# Autodesk Inventor assembly: OGRobotAssembly
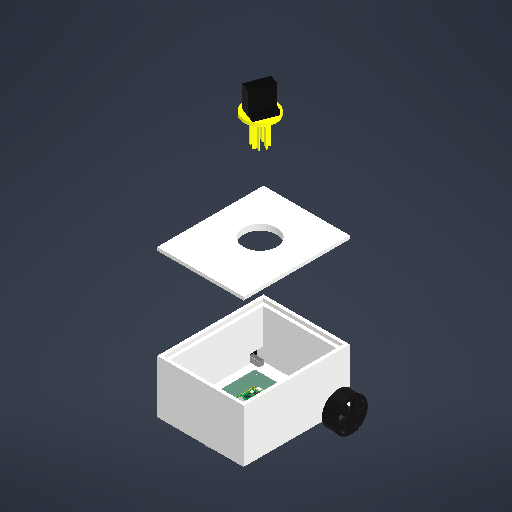
[picture p0: Inventor's stored thumbnail of the model, 512x512]
Saved by Autodesk Inventor 2027 (Build 310192060, 192F)
## iProperties
Created: 2026-07-04
Part Number: OGRobotAssembly
Document SubType Name: Assembly
Designer: machnach0
Author: machnach0
## Documents named in this file (9)
- C:\Users\machnach0\Documents\Inventor\Stardance Design Challenge\OGRobotAssembly.iam
- C:\Users\machnach0\Documents\Inventor\Stardance Design Challenge\OGRobotBase.ipt
- C:\Users\machnach0\Documents\Inventor\Stardance Design Challenge\OGRobotRoof.ipt
- C:\Users\machnach0\Documents\Inventor\Stardance Design Challenge\OGPlatform.ipt
- C:\Users\machnach0\Documents\Inventor\Stardance Design Challenge\OGWheel.ipt
- C:\Users\machnach0\Documents\Inventor\Stardance Design Challenge\OGGearMotor.ipt
- C:\Users\machnach0\Documents\Inventor\Stardance Design Challenge\OGCasterWheel.ipt
- C:\Users\machnach0\Documents\Inventor\Stardance Design Challenge\OGPCB.ipt
- C:\Users\machnach0\Documents\Inventor\Stardance Design Challenge\OGLiDAR.ipt
## Components (10 placed, 8 different names)
1. OGRobotBase:1 — Mate:1, Mate:2, Mate:9, Mate:10, Mate:11, Mate:12, Mate:13, Mate:14, Mate:15, Mate:16, Mate:17, Mate:18
2. OGRobotRoof:1 — Mate:1, Mate:2, Mate:4
3. OGPlatform:1 — Mate:4, Mate:19, Mate:20, Mate:21
4. OGWheel:1 — Mate:5, Mate:6, Mate:10
5. OGGearMotor:1 — Mate:5, Mate:6, Mate:9, Mate:11
6. OGWheel:2 — Mate:14
7. OGGearMotor:2 — Mate:12, Mate:13
8. OGCasterWheel:1 — Mate:15, Mate:16, Mate:17
9. OGPCB:1 — Mate:18
10. OGLiDAR:1 — Mate:19, Mate:20, Mate:21
## Relationships (20: Mate 20)
- Mate:1 (1.27 mm): OGRobotBase:1 ↔ OGRobotRoof:1
- Mate:2 (1.27 mm): OGRobotBase:1 ↔ OGRobotRoof:1
- Mate:4: OGRobotRoof:1 ↔ OGPlatform:1
- Mate:5: OGWheel:1 ↔ OGGearMotor:1
- Mate:6: OGWheel:1 ↔ OGGearMotor:1
- [Mate]: OGWheel:2 ↔ OGGearMotor:2
- [Mate]: OGWheel:2 ↔ OGGearMotor:2
- Mate:9 (6.731 mm): OGRobotBase:1 ↔ OGGearMotor:1
- Mate:10 (2.54 mm): OGRobotBase:1 ↔ OGWheel:1
- Mate:11 (2.54 mm): OGRobotBase:1 ↔ OGGearMotor:1
- Mate:12 (6.731 mm): OGRobotBase:1 ↔ OGGearMotor:2
- Mate:13 (2.54 mm): OGRobotBase:1 ↔ OGGearMotor:2
- Mate:14 (2.54 mm): OGRobotBase:1 ↔ OGWheel:2
- Mate:15: OGRobotBase:1 ↔ OGCasterWheel:1
- Mate:16 (-82.55 mm): OGRobotBase:1 ↔ OGCasterWheel:1
- Mate:17 (-25.4 mm): OGRobotBase:1 ↔ OGCasterWheel:1
- Mate:18: OGRobotBase:1 ↔ OGPCB:1
- Mate:19: OGPlatform:1 ↔ OGLiDAR:1
- Mate:20 (-21.59 mm): OGPlatform:1 ↔ OGLiDAR:1
- Mate:21 (-21.59 mm): OGPlatform:1 ↔ OGLiDAR:1
## Named parameters: d11_d9 = 0 mm, d12_d10 = 0 mm
